# Autodesk Inventor assembly: Assembly1 grab cad
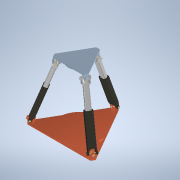
[picture p0: Inventor's stored thumbnail of the model, 180x180]
Saved by Autodesk Inventor 2020 (Build 240168000, 168)
## iProperties
Created: 2020-12-13
Part Number: Assembly1 grab cad
Document SubType Name: Assembly
Designer: Vikki
Author: Vikki
## Documents named in this file (7)
- D:\borewell rescuebot\pll manipulator files\sps manipulator\Assembly1 grab cad.iam
- D:\borewell rescuebot\2020 bot\actor_base_CATPart.ipt
- D:\borewell rescuebot\2020 bot\Ass.ipt
- D:\borewell rescuebot\2020 bot\base_CATPart.ipt
- D:\borewell rescuebot\2020 bot\cardan.ipt
- D:\borewell rescuebot\2020 bot\extension_CATPart.ipt
- D:\borewell rescuebot\2020 bot\upper_base_CAT.ipt
## Components (15 placed, 6 different names)
1. Ass:1
2. base_CATPart:1 — Mate:28, Mate:29, Mate:38, Mate:39, Mate:48, Mate:49, Mate:52
3. upper_base_CAT:1 — Mate:30, Mate:31, Mate:40, Mate:41, Mate:50, Mate:51, Mate:52
4. actor_base_CATPart:3 — Mate:26, Mate:27
5. cardan:5 — Mate:26, Mate:27, Mate:28, Mate:29
6. extension_CATPart:3
7. cardan:6 — Mate:30, Mate:31
8. actor_base_CATPart:4
9. cardan:7 — Mate:38, Mate:39
10. extension_CATPart:4
11. cardan:8 — Mate:40, Mate:41
12. actor_base_CATPart:5
13. cardan:9 — Mate:48, Mate:49
14. extension_CATPart:5
15. cardan:10 — Mate:50, Mate:51
## Relationships (31: Mate 31)
- [Mate]: actor_base_CATPart:3 ↔ extension_CATPart:3
- [Mate]: actor_base_CATPart:3 ↔ extension_CATPart:3
- [Mate]: extension_CATPart:3 ↔ cardan:6
- [Mate]: extension_CATPart:3 ↔ cardan:6
- Mate:26: actor_base_CATPart:3 ↔ cardan:5
- Mate:27: actor_base_CATPart:3 ↔ cardan:5
- Mate:28: base_CATPart:1 ↔ cardan:5
- Mate:29: base_CATPart:1 ↔ cardan:5
- Mate:30: upper_base_CAT:1 ↔ cardan:6
- Mate:31: upper_base_CAT:1 ↔ cardan:6
- [Mate]: actor_base_CATPart:4 ↔ extension_CATPart:4
- [Mate]: actor_base_CATPart:4 ↔ extension_CATPart:4
- [Mate]: extension_CATPart:4 ↔ cardan:8
- [Mate]: extension_CATPart:4 ↔ cardan:8
- [Mate]: actor_base_CATPart:4 ↔ cardan:7
- [Mate]: actor_base_CATPart:4 ↔ cardan:7
- Mate:38: base_CATPart:1 ↔ cardan:7
- Mate:39: base_CATPart:1 ↔ cardan:7
- Mate:40: upper_base_CAT:1 ↔ cardan:8
- Mate:41: upper_base_CAT:1 ↔ cardan:8
- [Mate]: actor_base_CATPart:5 ↔ extension_CATPart:5
- [Mate]: actor_base_CATPart:5 ↔ extension_CATPart:5
- [Mate]: extension_CATPart:5 ↔ cardan:10
- [Mate]: extension_CATPart:5 ↔ cardan:10
- [Mate]: actor_base_CATPart:5 ↔ cardan:9
- [Mate]: actor_base_CATPart:5 ↔ cardan:9
- Mate:48: base_CATPart:1 ↔ cardan:9
- Mate:49: base_CATPart:1 ↔ cardan:9
- Mate:50: upper_base_CAT:1 ↔ cardan:10
- Mate:51: upper_base_CAT:1 ↔ cardan:10
- Mate:52: base_CATPart:1 ↔ upper_base_CAT:1
## Named parameters: d23_d9 = 0 mm, d24_d10 = 0 mm, d25_d11 = 0 mm, d26_d12 = 0 mm, d37_d23_d9 = 0 mm, d38_d24_d10 = 0 mm, d39_d25_d11 = 0 mm, d40_d26_d12 = 0 mm, d41_d31 = 0 mm, d42_d32 = 0 mm, d47_d23_d9 = 0 mm, d48_d24_d10 = 0 mm, d49_d25_d11 = 0 mm, d50_d26_d12 = 0 mm, d51_d31 = 0 mm, d52_d32 = 0 mm
